# Autodesk Inventor assembly: guide wheel
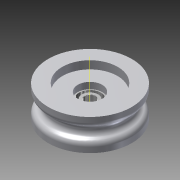
[picture p0: Inventor's stored thumbnail of the model, 180x180]
Saved by Autodesk Inventor 2013 (Build 170138000, 138)
## iProperties
Created: 2012-11-22
Part Number: guide wheel
Document SubType Name: Assembly
Designer: Nico
Author: Nico
## Documents named in this file (4)
- D:\Documents\Inventor\Coil winder\IAM files\guide wheel.iam
- D:\Documents\Inventor\Coil winder\IPT files\guidance wheel.ipt
- D:\Documents\Inventor\Content Center Files\R2013\en-US\ISO 1224 (I) M\ISO 1224 - 39 - 3 x 8 x 4.ipt
- D:\Documents\Inventor\Coil winder\IPT files\Bearring cap 8mm.ipt
## Components (3 placed, 3 different names)
1. guidance wheel:1 — Mate:1, Mate:2, Mate:3, Mate:4
2. ISO 1224 (I) (Metric) 39 - 3 x 8 x 4:1 — Mate:1, Mate:2
3. Bearring cap 8mm:1 — Mate:3, Mate:4
## Relationships (4: Mate 4)
- Mate:1: guidance wheel:1 ↔ ISO 1224 (I) (Metric) 39 - 3 x 8 x 4:1
- Mate:2: guidance wheel:1 ↔ ISO 1224 (I) (Metric) 39 - 3 x 8 x 4:1
- Mate:3: guidance wheel:1 ↔ Bearring cap 8mm:1
- Mate:4: guidance wheel:1 ↔ Bearring cap 8mm:1
